# Autodesk Inventor assembly: Roller Assembly
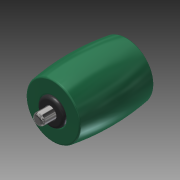
[picture p0: Inventor's stored thumbnail of the model, 180x180]
Saved by Autodesk Inventor 2016 (Build 200138000, 138)
## iProperties
Company: Bots 'n' Stuff
Created: 2014-01-10
Vendor: VEX Robotics, Inc.
Document SubType Name: Assembly
Designer: Jordan Kiesel
Catalog Web Link: http://vexrobotics.com/276-3526.html
Mass: 1.50123 g
Surface Area: 13.0181 cm^2
Volume: 1.03939 cm^3
Density: 1.44433 g/cm^3
Title: Roller Assembly
Author: Jordan Kiesel
## Documents named in this file (4)
- C:\Users\Jordan\Documents\Robotics\CAD\2015 BNS CAD Library (beta)\Motion\Wheels & Rollers\Reference Parts\3.25'' Omni-Directional Wheels\Reference Parts\Roller Assembly.iam
- C:\Users\Jordan\Documents\Robotics\CAD\2015 BNS CAD Library (beta)\Motion\Wheels & Rollers\Reference Parts\3.25'' Omni-Directional Wheels\Reference Parts\Reference Parts\Pin.ipt
- C:\Users\Jordan\Documents\Robotics\CAD\2015 BNS CAD Library (beta)\Motion\Wheels & Rollers\Reference Parts\3.25'' Omni-Directional Wheels\Reference Parts\Reference Parts\Roller.ipt
- C:\Users\Jordan\Documents\Robotics\CAD\2015 BNS CAD Library (beta)\Motion\Wheels & Rollers\Reference Parts\3.25'' Omni-Directional Wheels\Reference Parts\Reference Parts\Rubber.ipt
## Components (3 placed, 3 different names)
1. Pin:1 — Insert:1
2. Roller:1 — Insert:1, Insert:2
3. Rubber:1 — Insert:2
## Relationships (2: Insert 2)
- Insert:1 (2.275 mm): Pin:1 ↔ Roller:1
- Insert:2 (0.5 mm): Roller:1 ↔ Rubber:1
